# Autodesk Inventor assembly: FRC Arena 2013 (TEST VERSION)
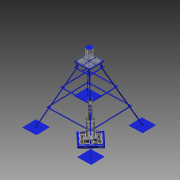
[picture p0: Inventor's stored thumbnail of the model, 180x180]
Saved by Autodesk Inventor 2013 (Build 170138000, 138)
## iProperties
Created: 2013-01-07
Part Number: FRC Arena 2013 (TEST VERSION)
Document SubType Name: Assembly
Designer: Phillip
Author: Phillip
## Documents named in this file (6)
- C:\Users\Arpan\Documents\GitHub\frc2013CAD\FIRST Arena 2013\FRC Arena 2013 (TEST VERSION).iam
- C:\Users\Arpan\Documents\GitHub\frc2013CAD\FIRST Arena 2013\Arena\Arena Base.ipt
- C:\Users\Arpan\Documents\GitHub\frc2013CAD\FIRST Arena 2013\Pyramid\GE-13017.iam
- C:\Users\Arpan\Documents\GitHub\frc2013CAD\FIRST Arena 2013\Playing Configuration Constraint.ipt
- C:\Users\Moses\Documents\GitHub\frc2013CAD\Robot Assembly V1.5 - 6 wheel - toughbox mini - 24x28.iam
- C:\Users\Arpan\Documents\GitHub\frc2013CAD\Robot Assembly - 6 wheel - toughbox mini - 26x28 official version.iam
## Components (5 placed, 5 different names)
1. Arena Base:1 — Mate:1, Mate:2, Angle:1, Mate:3, Angle:2, Flush:3, Mate:41, Mate:42
2. GE-13017:1 [sub-assembly] — Mate:1, Tangent:3, Tangent:4, Angle:3, Mate:44, Tangent:7, Tangent:8, Mate:45, Angle:4
3. Robot Assembly V1.5 - 6 wheel - toughbox mini - 24x28:1 [sub-assembly] — Mate:41, Mate:42, Tangent:3, Tangent:4, Tangent:5, Tangent:6, Angle:3, Mate:43, Tangent:7, Tangent:8
4. Playing Configuration Constraint:1 — Tangent:5, Tangent:6, Mate:43
5. Robot Assembly - 6 wheel - toughbox mini - 26x28 official version:1 [sub-assembly] — Mate:45, Angle:4
## Relationships (21: Mate 8, Tangent 6, Angle 4, Flush 3)
- Mate:1: Arena Base:1 ↔ GE-13017:1
- Mate:2: Arena Base:1
- Angle:1 (0 deg): Arena Base:1
- Flush:1 (2743.2 mm)
- Mate:3: Arena Base:1
- Angle:2 (0 deg): Arena Base:1
- Flush:2 (-2743.2 mm)
- Flush:3: Arena Base:1
- Mate:41 (1600.2 mm): Arena Base:1 ↔ Robot Assembly V1.5 - 6 wheel - toughbox mini - 24x28:1
- Mate:42 (1600.2 mm): Arena Base:1 ↔ Robot Assembly V1.5 - 6 wheel - toughbox mini - 24x28:1
- Tangent:3 (50.8 mm): GE-13017:1 ↔ Robot Assembly V1.5 - 6 wheel - toughbox mini - 24x28:1
- Tangent:4 (50.8 mm): GE-13017:1 ↔ Robot Assembly V1.5 - 6 wheel - toughbox mini - 24x28:1
- Tangent:5: Robot Assembly V1.5 - 6 wheel - toughbox mini - 24x28:1 ↔ Playing Configuration Constraint:1
- Tangent:6: Robot Assembly V1.5 - 6 wheel - toughbox mini - 24x28:1 ↔ Playing Configuration Constraint:1
- Angle:3 (45 deg): GE-13017:1 ↔ Robot Assembly V1.5 - 6 wheel - toughbox mini - 24x28:1
- Mate:43 (-76.2 mm): Robot Assembly V1.5 - 6 wheel - toughbox mini - 24x28:1 ↔ Playing Configuration Constraint:1
- Mate:44: GE-13017:1
- Tangent:7: GE-13017:1 ↔ Robot Assembly V1.5 - 6 wheel - toughbox mini - 24x28:1
- Tangent:8: GE-13017:1 ↔ Robot Assembly V1.5 - 6 wheel - toughbox mini - 24x28:1
- Mate:45: GE-13017:1 ↔ Robot Assembly - 6 wheel - toughbox mini - 26x28 official version:1
- Angle:4 (0 deg): GE-13017:1 ↔ Robot Assembly - 6 wheel - toughbox mini - 26x28 official version:1
